# Autodesk Inventor assembly: TR2 Arm
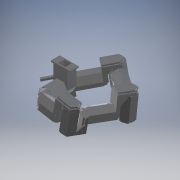
[picture p0: Inventor's stored thumbnail of the model, 180x180]
Saved by Autodesk Inventor 2017 (Build 210142000, 142)
## iProperties
Created: 2018-10-11
Part Number: TR2 Arm
Document SubType Name: Assembly
Designer: Zach
Author: Zach
## Documents named in this file (11)
- C:\Users\Dell\Documents\GitHub\tr2\Arm\Arm.iam
- C:\Users\Dell\Documents\GitHub\tr2\Arm\TARM01.ipt
- C:\Users\Dell\Documents\GitHub\tr2\Arm Actuator\Arm Actuator.iam
- C:\Users\Dell\Documents\GitHub\tr2\Arm\TARM02.ipt
- C:\Users\Dell\Documents\GitHub\tr2\Arm\TARM03.ipt
- C:\Users\Dell\Documents\GitHub\tr2\Arm\TARM04.ipt
- C:\Users\Dell\Documents\GitHub\tr2\Arm\TARM05.ipt
- C:\Users\Dell\Documents\GitHub\tr2\Arm\TARM06.ipt
- C:\Users\Dell\Documents\GitHub\tr2\Arm\TARM07.ipt
- C:\Users\Dell\Documents\GitHub\tr2\Arm\TARM08.ipt
- C:\Users\Dell\Documents\GitHub\tr2\Gripper\Gripper.iam
## Components (29 placed, 10 different names)
1. TARM01:1 — Mate:11, Mate:117, Mate:118
2. TARM02:1 — Mate:13, Mate:20, Mate:106, Mate:108, Mate:109, Mate:110, Mate:119, Mate:120
3. TARM03:1 — Mate:20, Mate:23, Mate:24, Mate:63, Mate:64, Mate:65, Mate:68, Mate:100, Mate:119, Mate:120
4. TARM03:2 — Mate:33, Mate:69, Mate:70, Mate:77, Mate:102, Mate:123, Mate:124
5. Arm Actuator:1 [sub-assembly] — Mate:11, Mate:13, Mate:106, Mate:117, Mate:118
6. Arm Actuator:2 [sub-assembly] — Mate:23, Mate:24, Mate:45, Mate:114, Mate:121, Mate:122
7. Arm Actuator:3 [sub-assembly] — Mate:33, Mate:48, Mate:113, Mate:123, Mate:124
8. Arm Actuator:4 [sub-assembly] — Mate:50, Mate:125, Mate:126
9. Arm Actuator:5 [sub-assembly] — Mate:40, Mate:53, Mate:112, Mate:127, Mate:128
10. Arm Actuator:6 [sub-assembly] — Mate:55, Mate:129, Mate:130
11. Arm Actuator:7 [sub-assembly] — Mate:58, Mate:111, Mate:116
12. TARM03:3 — Mate:40, Mate:72, Mate:73, Mate:80, Mate:104, Mate:127, Mate:128
13. TARM04:1 — Mate:45, Mate:48, Mate:88, Mate:89, Mate:92, Mate:101, Mate:113, Mate:114, Mate:121, Mate:122
14. TARM04:2 — Mate:50, Mate:53, Mate:84, Mate:86, Mate:93, Mate:95, Mate:96, Mate:103, Mate:112, Mate:125, Mate:126
15. TARM04:3 — Mate:55, Mate:58, Mate:81, Mate:83, Mate:97, Mate:98, Mate:99, Mate:105, Mate:111, Mate:129, Mate:130
16. TARM05:1 — Mate:65, Mate:66, Mate:100
17. TARM06:1 — Mate:63, Mate:64, Mate:66, Mate:68
18. TARM05:2 — Mate:69, Mate:70, Mate:75, Mate:76, Mate:102
19. TARM05:3 — Mate:72, Mate:73, Mate:78, Mate:79, Mate:104
20. TARM06:2 — Mate:75, Mate:76, Mate:77
21. TARM06:3 — Mate:78, Mate:79, Mate:80
22. TARM05:4 — Mate:81, Mate:83, Mate:105
23. TARM05:5 — Mate:84, Mate:86, Mate:94, Mate:95, Mate:103
24. TARM05:6 — Mate:88, Mate:89, Mate:90, Mate:91, Mate:101
25. TARM07:1 — Mate:90, Mate:91, Mate:92
26. TARM07:2 — Mate:93, Mate:94, Mate:96
27. TARM07:3 — Mate:97, Mate:98, Mate:99
28. TARM08:1 — Mate:108, Mate:109, Mate:110
29. Gripper:1 [sub-assembly] — Mate:116
## Relationships (77: Mate 77)
- Mate:11: TARM01:1 ↔ Arm Actuator:1
- Mate:13: TARM02:1 ↔ Arm Actuator:1
- Mate:20: TARM02:1 ↔ TARM03:1
- Mate:23: TARM03:1 ↔ Arm Actuator:2
- Mate:24: TARM03:1 ↔ Arm Actuator:2
- [Mate]: TARM03:2 ↔ Arm Actuator:4
- [Mate]: TARM03:2 ↔ Arm Actuator:4
- Mate:33: TARM03:2 ↔ Arm Actuator:3
- [Mate]: Arm Actuator:6 ↔ TARM03:3
- [Mate]: Arm Actuator:6 ↔ TARM03:3
- Mate:40: Arm Actuator:5 ↔ TARM03:3
- Mate:45: Arm Actuator:2 ↔ TARM04:1
- Mate:48: Arm Actuator:3 ↔ TARM04:1
- Mate:50: Arm Actuator:4 ↔ TARM04:2
- Mate:53: Arm Actuator:5 ↔ TARM04:2
- Mate:55: Arm Actuator:6 ↔ TARM04:3
- Mate:58: Arm Actuator:7 ↔ TARM04:3
- Mate:63: TARM03:1 ↔ TARM06:1
- Mate:64: TARM03:1 ↔ TARM06:1
- Mate:65: TARM03:1 ↔ TARM05:1
- Mate:66: TARM05:1 ↔ TARM06:1
- Mate:68: TARM03:1 ↔ TARM06:1
- Mate:69: TARM03:2 ↔ TARM05:2
- Mate:70: TARM03:2 ↔ TARM05:2
- Mate:72: TARM03:3 ↔ TARM05:3
- Mate:73: TARM03:3 ↔ TARM05:3
- Mate:75: TARM05:2 ↔ TARM06:2
- Mate:76: TARM05:2 ↔ TARM06:2
- Mate:77: TARM03:2 ↔ TARM06:2
- Mate:78: TARM05:3 ↔ TARM06:3
- Mate:79: TARM05:3 ↔ TARM06:3
- Mate:80: TARM03:3 ↔ TARM06:3
- Mate:81: TARM04:3 ↔ TARM05:4
- Mate:83: TARM04:3 ↔ TARM05:4
- Mate:84: TARM04:2 ↔ TARM05:5
- Mate:86: TARM04:2 ↔ TARM05:5
- Mate:88: TARM04:1 ↔ TARM05:6
- Mate:89: TARM04:1 ↔ TARM05:6
- Mate:90: TARM05:6 ↔ TARM07:1
- Mate:91: TARM05:6 ↔ TARM07:1
- Mate:92: TARM04:1 ↔ TARM07:1
- Mate:93: TARM04:2 ↔ TARM07:2
- Mate:94: TARM05:5 ↔ TARM07:2
- Mate:95: TARM04:2 ↔ TARM05:5
- Mate:96: TARM04:2 ↔ TARM07:2
- Mate:97: TARM04:3 ↔ TARM07:3
- Mate:98: TARM04:3 ↔ TARM07:3
- Mate:99: TARM04:3 ↔ TARM07:3
- Mate:100: TARM03:1 ↔ TARM05:1
- Mate:101: TARM04:1 ↔ TARM05:6
- Mate:102: TARM03:2 ↔ TARM05:2
- Mate:103: TARM04:2 ↔ TARM05:5
- Mate:104: TARM03:3 ↔ TARM05:3
- Mate:105: TARM04:3 ↔ TARM05:4
- Mate:106: TARM02:1 ↔ Arm Actuator:1
- Mate:108: TARM02:1 ↔ TARM08:1
- Mate:109: TARM02:1 ↔ TARM08:1
- Mate:110: TARM02:1 ↔ TARM08:1
- Mate:111: Arm Actuator:7 ↔ TARM04:3
- Mate:112: Arm Actuator:5 ↔ TARM04:2
- Mate:113: Arm Actuator:3 ↔ TARM04:1
- Mate:114: Arm Actuator:2 ↔ TARM04:1
- Mate:116: Arm Actuator:7 ↔ Gripper:1
- Mate:117: TARM01:1 ↔ Arm Actuator:1
- Mate:118: TARM01:1 ↔ Arm Actuator:1
- Mate:119: TARM02:1 ↔ TARM03:1
- Mate:120: TARM02:1 ↔ TARM03:1
- Mate:121: Arm Actuator:2 ↔ TARM04:1
- Mate:122: Arm Actuator:2 ↔ TARM04:1
- Mate:123: TARM03:2 ↔ Arm Actuator:3
- Mate:124: TARM03:2 ↔ Arm Actuator:3
- Mate:125: Arm Actuator:4 ↔ TARM04:2
- Mate:126: Arm Actuator:4 ↔ TARM04:2
- Mate:127: Arm Actuator:5 ↔ TARM03:3
- Mate:128: Arm Actuator:5 ↔ TARM03:3
- Mate:129: Arm Actuator:6 ↔ TARM04:3
- Mate:130: Arm Actuator:6 ↔ TARM04:3
## Named parameters: d86_d78 = 0 mm, d87_d79 = 0 mm, d93_d86_d78 = 0 mm, d94_d87_d79 = 0 mm
